# Autodesk Inventor assembly: Box_assembly
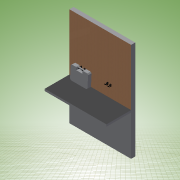
[picture p0: Inventor's stored thumbnail of the model, 180x180]
Saved by Autodesk Inventor 2017 (Build 210142000, 142)
## iProperties
Created: 2018-06-04
Part Number: Box_assembly
Document SubType Name: Assembly
Designer: Spark Electronics
Author: Spark Electronics
## Documents named in this file (6)
- C:\Users\Owner\Documents\SPARK RESEARCH\Projects\Organization\Divider Boxes\Box_assembly.iam
- C:\Users\Owner\Documents\SPARK RESEARCH\Projects\Organization\Divider Boxes\Wall_desk.ipt
- C:\Users\Owner\Documents\SPARK RESEARCH\Projects\Organization\Divider Boxes\Divider_box.ipt
- C:\Users\Owner\Documents\SPARK RESEARCH\Projects\Organization\Divider Boxes\wall_hook.ipt
- C:\Users\Owner\Documents\SPARK RESEARCH\Projects\Organization\Divider Boxes\Wall_mount.ipt
- C:\Users\Owner\Documents\SPARK RESEARCH\Projects\Organization\Divider Boxes\drill guide.ipt
## Components (9 placed, 5 different names)
1. Wall_desk:1 — Mate:1, Mate:2, Flush:6, Mate:11, Mate:12, Flush:8
2. Divider_box:1 — Mate:5, Mate:8, Mate:21, Mate:24
3. wall_hook:1 — Flush:5, Mate:8, Mate:13, Mate:14, Mate:21, Flush:8
4. wall_hook:2 — Flush:5, Mate:5, Flush:6, Mate:16, Mate:22, Mate:23, Mate:24
5. wall_hook:3 — Mate:2
6. wall_hook:4 — Mate:1
7. Wall_mount:1 — Mate:12, Flush:7, Mate:13, Mate:14, Mate:18, Mate:19, Mate:20
8. Wall_mount:2 — Mate:11, Flush:7, Mate:16, Mate:17, Mate:22, Mate:23
9. drill guide:1 — Mate:17, Mate:18, Mate:19, Mate:20
## Relationships (21: Mate 17, Flush 4)
- Mate:1: Wall_desk:1 ↔ wall_hook:4
- Mate:2: Wall_desk:1 ↔ wall_hook:3
- Flush:5: wall_hook:1 ↔ wall_hook:2
- Mate:5: Divider_box:1 ↔ wall_hook:2
- Mate:8: Divider_box:1 ↔ wall_hook:1
- Flush:6 (381 mm): Wall_desk:1 ↔ wall_hook:2
- Mate:11: Wall_desk:1 ↔ Wall_mount:2
- Mate:12: Wall_desk:1 ↔ Wall_mount:1
- Flush:7: Wall_mount:1 ↔ Wall_mount:2
- Mate:13 (0.1 mm): wall_hook:1 ↔ Wall_mount:1
- Mate:14 (0.1 mm): wall_hook:1 ↔ Wall_mount:1
- Mate:16: wall_hook:2 ↔ Wall_mount:2
- Mate:17: Wall_mount:2 ↔ drill guide:1
- Mate:18: Wall_mount:1 ↔ drill guide:1
- Mate:19: Wall_mount:1 ↔ drill guide:1
- Mate:20: Wall_mount:1 ↔ drill guide:1
- Mate:21 (25.4 mm): Divider_box:1 ↔ wall_hook:1
- Mate:22: wall_hook:2 ↔ Wall_mount:2
- Mate:23 (0.1016 mm): wall_hook:2 ↔ Wall_mount:2
- Flush:8 (-335.28 mm): Wall_desk:1 ↔ wall_hook:1
- Mate:24 (9.144 mm): Divider_box:1 ↔ wall_hook:2
